# Autodesk Inventor assembly: Assembly1
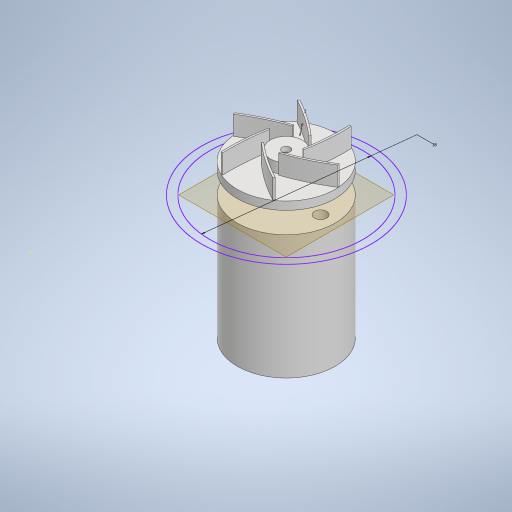
[picture p0: Inventor's stored thumbnail of the model, 512x512]
Saved by Autodesk Inventor 2023.1 (Build 271208000, 208)
## iProperties
Created: 2024-02-14
Part Number: Assembly1
Document SubType Name: Assembly
Designer: USER
Author: USER
## Documents named in this file (4)
- C:\Users\USER\Documents\WaterPump\Assembly1.iam
- C:\Users\USER\Documents\Vesters3DPrinter\UpperCrossGantryLowCost\Propeller.ipt
- C:\Users\USER\Documents\WaterPump\Motor.ipt
- C:\Users\USER\Documents\WaterPump\case.ipt
## Components (3 placed, 3 different names)
1. Propeller:1 — Insert:1
2. Motor:1 — Insert:1, Flush:1
3. case:1 — Flush:1
## Relationships (2: Insert 1, Flush 1)
- Insert:1: Propeller:1 ↔ Motor:1
- Flush:1: Motor:1 ↔ case:1
